# Autodesk Inventor assembly: Degrader_Assembly
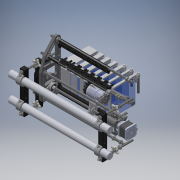
[picture p0: Inventor's stored thumbnail of the model, 180x180]
Saved by Autodesk Inventor 2019 (Build 230136000, 136)
## iProperties
Created: 2019-10-16
Part Number: Degrader_Assembly
Document SubType Name: Assembly
Designer: 19879326
Author: 19879326
## Documents named in this file (57)
- I:\Poster\CAD\CAD\Final\Degrader_Assembly.iam
- I:\Poster\CAD\CAD\Final\Mount\Mounting Rods.ipt
- I:\Poster\CAD\CAD\Final\Mount\Mount_Block.ipt
- I:\Poster\CAD\CAD\Final\Frame\Frame_Stepper_New.ipt
- I:\Poster\CAD\CAD\Final\Frame\Frame_Bearing_New.ipt
- I:\Poster\CAD\CAD\Final\Frame\Thread_Shaft_330mm.ipt
- I:\Poster\CAD\CAD\Final\Frame\300mm_Rod.ipt
- I:\Poster\CAD\CAD\Final\Mount\Mount_Thread.ipt
- I:\Poster\CAD\CAD\Final\Mount\M8_Nut.ipt
- I:\Poster\CAD\CAD\Final\Frame\Thread_Shaft_366mm.ipt
- I:\Poster\CAD\CAD\Final\Mount\Wing_Nut.ipt
- I:\Poster\CAD\CAD\Final\Mount\Frame_Mount.ipt
- I:\Poster\CAD\CAD\Final\Stepper Motor\Bearing.ipt
- I:\Poster\CAD\CAD\Final\Stepper Motor\Pillow_Stand.ipt
- I:\Poster\CAD\CAD\Final\Stepper Motor\Screw.ipt
- I:\Poster\CAD\CAD\Final\Stepper Motor\Stepper_Nema17.ipt
- I:\Poster\CAD\CAD\Final\Stepper Motor\Thread_Shaft.ipt
- I:\Poster\CAD\CAD\Final\Stepper Motor\Coupler.ipt
- I:\Poster\CAD\CAD\Final\DC motor\DC Gear.ipt
- I:\Poster\CAD\CAD\Final\DC motor\Frame_DC.ipt
- I:\Poster\CAD\CAD\Final\DC motor\Linear Bearing 8mm.ipt
- I:\Poster\CAD\CAD\Final\DC motor\DC_Motor.iam
- I:\Poster\CAD\CAD\Final\Sheet Holders\2mmFrame.ipt
- I:\Poster\CAD\CAD\Final\Sheet Holders\3mmFrame.ipt
- I:\Poster\CAD\CAD\Final\Sheet Holders\6mmFrame.ipt
- I:\Poster\CAD\CAD\Final\Sheet Holders\8mmFrame.ipt
- I:\Poster\CAD\CAD\Final\Sheet Holders\10mmFrame.ipt
- I:\Poster\CAD\CAD\Final\Sheet Holders\12mmFrame.ipt
- I:\Poster\CAD\CAD\Final\Sheet Holders\30mmFrame.ipt
- I:\Poster\CAD\CAD\Final\Sheet Holders\Spacer.ipt
- I:\Poster\CAD\CAD\Final\Switches\Roller_Switch._new.ipt
- I:\Poster\CAD\CAD\Final\Frame\M8_Nut.ipt
- I:\Poster\CAD\CAD\Final\Switches\30_Switch_Left.ipt
- I:\Poster\CAD\CAD\Final\Switches\30_Switch.ipt
- I:\Poster\CAD\CAD\Final\Switches\Switch holder_Right.ipt
- I:\Poster\CAD\CAD\Final\Switches\Switch holder_Left.ipt
- I:\Poster\CAD\CAD\Final\Switches\Roller_Spacer.ipt
- I:\Poster\CAD\CAD\Final\Switches\Roller_Spacer_P.ipt
- I:\Poster\CAD\CAD\Final\Switches\Roller_Switch _30_new.ipt
- I:\Poster\CAD\CAD\Final\Switches\Roller_Switch end.ipt
- I:\Poster\CAD\CAD\Final\Mount\Clamp_Mount.ipt
- I:\Poster\CAD\CAD\Final\Sheet Holders\Sheet_2mm.ipt
- I:\Poster\CAD\CAD\Final\Sheet Holders\Sheet_3mm.ipt
- I:\Poster\CAD\CAD\Final\Sheet Holders\Sheet_6mm.ipt
- I:\Poster\CAD\CAD\Final\Sheet Holders\Sheet_8mm.ipt
- I:\Poster\CAD\CAD\Final\Sheet Holders\Sheet_10mm.ipt
- I:\Poster\CAD\CAD\Final\Sheet Holders\Sheet_12mm.ipt
- I:\Poster\CAD\CAD\Final\Sheet Holders\Sheet_30mm.ipt
- I:\Poster\CAD\CAD\Final\Frame\Cap.ipt
- I:\Poster\CAD\CAD\Final\Sheet Holders\6mm Weight Clamp.ipt
- I:\Poster\CAD\CAD\Final\Sheet Holders\2mm_3mm Weight Clamp.ipt
- I:\Poster\CAD\CAD\Final\Sheet Holders\Weight_Thread_2mm.ipt
- I:\Poster\CAD\CAD\Final\Sheet Holders\Weight_Thread_3mm.ipt
- I:\Poster\CAD\CAD\Final\Sheet Holders\Weight_Thread_6mm.ipt
- I:\Poster\CAD\CAD\Final\Sheet Holders\frameClip.ipt
- I:\Poster\CAD\CAD\Final\DC motor\DC_Ring.ipt
- I:\Poster\CAD\CAD\Final\DC motor\Thread_Clip.ipt
## Components (143 placed, 55 different names)
1. Mounting Rods:1 — Mate:1, Mate:2, Mate:3, Flush:13, Mate:261, Mate:262, Mate:263, Mate:264
2. Mount_Block:1 — Mate:1, Flush:1, Mate:31, Mate:32, Mate:34, Mate:36, Mate:37, Mate:38, Mate:48, Mate:50, Flush:11, Flush:12, Flush:42, Flush:43, Mate:265
3. Mount_Block:2 — Mate:2, Mate:3, Flush:1, Mate:30, Mate:33, Mate:40, Mate:42, Mate:43, Mate:44, Mate:46, Mate:52, Flush:9, Flush:10, Flush:13, Flush:40, Flush:41
4. Frame_Bearing_New:1 — Mate:84, Mate:85, Mate:86, Mate:87, Mate:88, Flush:15, Flush:16, Flush:17, Flush:18, Flush:19, Mate:96, Mate:104, Mate:135, Mate:137, Mate:154, Mate:166, Mate:167, Mate:168, Mate:169, Mate:170, Mate:178, Mate:179, Mate:180, Mate:212, Mate:213, Mate:215, Mate:216, Mate:242, Angle:1, Mate:280, Mate:281, Mate:282, Mate:284, Mate:288
5. Frame_Stepper_New:1 — Mate:89, Mate:91, Mate:92, Mate:93, Mate:94, Mate:95, Mate:96, Mate:97, Mate:98, Mate:99, Mate:100, Mate:101, Mate:122, Mate:123, Mate:124, Mate:129, Mate:130, Mate:131, Mate:163, Mate:164, Mate:171, Mate:172, Mate:175, Mate:181, Mate:182, Mate:183, Mate:184, Mate:185, Mate:186, Mate:188, Mate:190, Mate:192, Mate:194, Flush:39, Mate:286, Mate:287, Mate:289, Mate:290, Mate:291
6. Mount_Thread:1 — Mate:30, Mate:41, Mate:53, Flush:9, Mate:79, Mate:114
7. Mount_Thread:2 — Mate:31, Mate:35, Mate:51, Flush:12, Mate:77, Mate:107, Mate:118
8. Mount_Thread:3 — Mate:32, Mate:39, Mate:49, Flush:11, Mate:81, Mate:120
9. Mount_Thread:4 — Mate:33, Mate:45, Mate:47, Flush:10, Mate:83, Mate:108, Mate:116
10. M8_Nut:1 — Mate:52, Mate:53
11. M8_Nut:2 — Mate:37, Mate:38, Mate:39
12. M8_Nut:3 — Mate:43, Mate:44, Mate:45
13. M8_Nut:4 — Mate:46, Mate:47
14. M8_Nut:5 — Mate:40, Mate:41, Mate:42
15. M8_Nut:6 — Mate:34, Mate:35, Mate:36
16. M8_Nut:7 — Mate:48, Mate:49
17. M8_Nut:8 — Mate:50, Mate:51
18. M8_Nut:9 — Mate:73, Mate:74, Mate:75, Mate:81
19. Wing_Nut:1 — Mate:73, Mate:74, Mate:75, Mate:110
20. M8_Nut:10 — Mate:70, Mate:71, Mate:72, Mate:79
21. Wing_Nut:2 — Mate:70, Mate:71, Mate:72, Mate:111
22. M8_Nut:11 — Mate:67, Mate:68, Mate:69, Mate:83
23. Wing_Nut:3 — Mate:67, Mate:68, Mate:69, Mate:112
24. M8_Nut:12 — Mate:64, Mate:65, Mate:66, Mate:77
25. Wing_Nut:4 — Mate:64, Mate:65, Mate:66, Mate:109
26. Thread_Shaft_330mm:1 — Mate:86, Flush:15, Mate:91, Mate:93, Mate:195, Mate:200, Mate:201, Mate:204, Mate:211, Mate:229, Mate:230, Mate:231, Mate:232, Mate:233, Mate:234
27. Thread_Shaft_366mm:1 — Mate:88, Flush:17, Mate:94, Mate:102, Mate:105, Mate:187, Mate:197, Mate:207, Mate:210
28. Thread_Shaft_330mm:2 — Mate:85, Flush:18, Mate:92, Mate:193, Mate:199, Mate:203, Mate:205, Mate:241, Mate:243, Mate:246, Mate:249, Mate:250, Mate:251, Mate:252, Mate:253, Mate:259, Mate:332
29. Thread_Shaft_366mm:2 — Mate:87, Flush:19, Mate:95, Mate:103, Mate:106, Mate:191, Mate:198, Mate:202, Mate:206
30. Thread_Shaft_330mm:3 — Mate:84, Flush:16, Mate:89, Mate:189, Mate:196, Mate:208, Mate:209, Mate:214, Mate:217, Mate:218, Mate:219, Mate:220, Mate:221, Mate:222
31. 300mm_Rod:1 — Mate:97, Mate:99, Mate:155, Mate:156, Mate:157, Mate:158, Mate:159, Mate:160, Mate:161, Mate:162, Mate:285
32. 300mm_Rod:2 — Mate:98, Mate:100, Mate:146, Mate:283
33. Frame_Mount:1 — Mate:101, Mate:102, Mate:103, Mate:108, Mate:111, Mate:112, Mate:113, Mate:115, Mate:173, Mate:174
34. Frame_Mount:2 — Mate:104, Mate:105, Mate:106, Mate:107, Mate:109, Mate:110, Mate:117, Mate:119, Mate:176, Mate:177, Mate:265
35. M8_Nut:13 — Mate:113, Mate:114
36. M8_Nut:14 — Mate:119, Mate:120
37. M8_Nut:15 — Mate:115, Mate:116
38. M8_Nut:16 — Mate:117, Mate:118
39. Bearing:1 — Mate:132, Mate:133, Mate:134
40. Pillow_Stand:1 — Mate:129, Mate:130, Mate:131, Mate:132, Mate:133
41. Screw:1 — Mate:142, Mate:143, Mate:144, Mate:147
42. Stepper_Nema17:1 — Mate:122, Mate:123, Mate:124, Mate:125, Mate:126
43. Thread_Shaft:1 — Mate:127, Mate:128, Mate:134, Mate:136, Mate:147
44. Bearing:2 — Mate:135, Mate:136, Mate:137
45. Coupler:1 — Mate:125, Mate:126, Mate:127, Mate:128
46. DC Gear:1 — Mate:145, Flush:21
47. Frame_DC:1 — Mate:138, Flush:20, Mate:139, Mate:140, Mate:142, Mate:143, Mate:144, Mate:292
48. Linear Bearing 8mm:1 — Mate:138, Flush:20, Mate:146
49. DC_Motor:1 [sub-assembly] — Mate:139, Mate:140, Mate:145, Flush:21, Mate:292, Mate:331
50. 2mmFrame:1 — Mate:148, Mate:161, Flush:39, Flush:49, Mate:266, Mate:267, Flush:51, Mate:293, Mate:294, Angle:2, Mate:295, Mate:296, Angle:3, Flush:66, Flush:75, Flush:77, Flush:78
51. 3mmFrame:1 — Mate:148, Mate:149, Mate:160, Flush:48, Flush:49, Mate:268, Mate:269, Flush:52, Mate:297, Mate:298, Mate:299, Mate:300, Angle:4, Angle:5, Flush:67, Flush:76, Flush:79, Flush:80
52. 6mmFrame:1 — Mate:149, Mate:150, Mate:159, Flush:47, Flush:48, Mate:270, Mate:271, Flush:53, Mate:301, Mate:302, Angle:6, Mate:303, Mate:304, Angle:7, Mate:330, Flush:81, Flush:82
53. 8mmFrame:1 — Mate:150, Mate:151, Mate:158, Flush:46, Flush:47, Mate:272, Mate:273, Flush:54, Mate:329, Flush:68, Flush:72, Flush:83, Flush:84
54. 10mmFrame:1 — Mate:151, Mate:152, Mate:157, Flush:45, Flush:46, Mate:274, Mate:275, Flush:55, Mate:328, Flush:69, Flush:71, Flush:85, Flush:86
55. 12mmFrame:1 — Mate:152, Mate:153, Mate:156, Flush:44, Flush:45, Mate:276, Mate:277, Flush:56, Mate:327, Flush:70, Flush:73, Flush:87, Flush:88
56. 30mmFrame:1 — Mate:153, Mate:154, Mate:155, Flush:44, Mate:278, Mate:279, Flush:57, Flush:64, Mate:312, Flush:65, Mate:326, Flush:74
57. Spacer:1 — Mate:162, Mate:163, Mate:164
58. M8_Nut:17 — Mate:178, Mate:199
59. M8_Nut:18 — Mate:175, Mate:208
60. M8_Nut:19 — Mate:174, Mate:207
61. M8_Nut:20 — Mate:172, Mate:205
62. M8_Nut:21 — Mate:173, Mate:206
63. M8_Nut:22 — Mate:181, Mate:194, Mate:195
64. M8_Nut:23 — Mate:179, Mate:200
65. M8_Nut:24 — Mate:185, Mate:186, Mate:187
66. M8_Nut:25 — Mate:180, Mate:196
67. M8_Nut:26 — Mate:170, Mate:210
68. M8_Nut:27 — Mate:177, Mate:198
69. M8_Nut:28 — Mate:169, Mate:209
70. M8_Nut:29 — Mate:168, Mate:203
71. M8_Nut:30 — Mate:167, Mate:202
72. M8_Nut:31 — Mate:166, Mate:201
73. M8_Nut:32 — Mate:184, Mate:188, Mate:189
74. M8_Nut:33 — Mate:183, Mate:190, Mate:191
75. M8_Nut:34 — Mate:182, Mate:192, Mate:193
76. M8_Nut:35 — Mate:176, Mate:197
77. M8_Nut:36 — Mate:171, Mate:204
78. 30_Switch_Left:1 — Mate:211, Mate:212, Mate:213, Mate:235, Flush:32
79. 30_Switch:1 — Mate:214, Mate:215, Mate:216, Mate:223, Flush:27
80. Switch holder_Right:1 — Mate:221, Mate:226, Mate:227, Flush:23, Flush:24
81. Switch holder_Right:2 — Mate:220, Mate:228, Flush:22
82. Switch holder_Right:3 — Mate:222, Mate:225, Mate:226, Flush:24, Flush:25
83. Switch holder_Right:4 — Mate:219, Mate:227, Mate:228, Flush:22, Flush:23
84. Switch holder_Right:5 — Mate:218, Mate:224, Mate:225, Flush:25, Flush:26
85. Switch holder_Right:6 — Mate:217, Mate:223, Mate:224, Flush:26, Flush:27
86. Switch holder_Left:1 — Mate:229, Mate:235, Mate:236, Flush:31, Flush:32
87. Switch holder_Left:2 — Mate:230, Mate:236, Mate:237, Flush:30, Flush:31
88. Switch holder_Left:3 — Mate:231, Mate:237, Mate:238, Flush:29, Flush:30
89. Switch holder_Left:4 — Mate:232, Mate:238, Mate:239, Flush:29, Flush:50
90. Switch holder_Left:5 — Mate:233, Mate:239, Mate:240, Flush:28, Flush:50
91. Switch holder_Left:6 — Mate:234, Mate:240, Flush:28
92. Roller_Spacer:1 — Mate:241, Mate:242, Angle:1, Mate:244, Mate:245
93. Roller_Spacer_P:1 — Mate:243, Mate:244, Mate:245, Mate:247, Mate:248
94. Roller_Switch._new:2 — Mate:252, Mate:256, Mate:257, Flush:35, Flush:36
95. Roller_Switch._new:3 — Mate:251, Mate:255, Mate:256, Flush:34, Flush:35
96. Roller_Switch._new:4 — Mate:250, Mate:254, Mate:255, Flush:33, Flush:34
97. Roller_Switch._new:5 — Mate:249, Mate:257, Mate:258, Flush:36, Flush:37
98. Roller_Switch._new:6 — Mate:253, Mate:258, Mate:260, Flush:37, Flush:38
99. Roller_Switch _30_new:1 — Mate:246, Mate:247, Mate:248, Mate:254, Flush:33
100. Roller_Switch end:1 — Mate:259, Mate:260, Flush:38, Angle:8
101. Clamp_Mount:1 — Mate:261, Flush:41
102. Clamp_Mount:2 — Mate:262, Flush:42
103. Clamp_Mount:3 — Mate:263, Flush:40
104. Clamp_Mount:4 — Mate:264, Flush:43
105. Sheet_2mm:1 — Mate:266, Mate:267, Flush:51, Mate:318, Mate:319
106. Sheet_3mm:1 — Mate:268, Mate:269, Flush:52, Mate:317, Mate:323
107. Sheet_6mm:1 — Mate:270, Mate:271, Flush:53, Mate:316, Mate:325
108. Sheet_8mm:1 — Mate:272, Mate:273, Flush:54, Mate:315, Mate:322
109. Sheet_10mm:1 — Mate:274, Mate:275, Flush:55, Mate:314, Mate:324
110. Sheet_12mm:1 — Mate:276, Mate:277, Flush:56, Mate:313, Mate:321
111. Sheet_30mm:1 — Mate:278, Mate:279, Flush:57, Mate:311, Mate:320
112. Cap:1 — Mate:285, Mate:286, Mate:287
113. Cap:2 — Mate:280, Mate:281, Mate:282
114. Cap:3 — Mate:283, Mate:284, Mate:288
115. Cap:4 — Mate:289, Mate:290, Mate:291
116. 6mm Weight Clamp:1 — Mate:303, Mate:304, Angle:7, Mate:306, Flush:63
117. 6mm Weight Clamp:2 — Mate:301, Mate:302, Angle:6, Mate:305, Flush:60
118. 2mm_3mm Weight Clamp:1 — Mate:293, Mate:294, Angle:2, Mate:310, Flush:58
119. 2mm_3mm Weight Clamp:2 — Mate:295, Mate:296, Angle:3, Mate:309, Flush:61
120. 2mm_3mm Weight Clamp:3 — Mate:299, Mate:300, Angle:4, Mate:307, Flush:62
121. 2mm_3mm Weight Clamp:4 — Mate:297, Mate:298, Angle:5, Mate:308, Flush:59
122. Weight_Thread_2mm:1 — Mate:310, Flush:58
123. Weight_Thread_3mm:1 — Mate:307, Flush:62
124. Weight_Thread_6mm:1 — Mate:306, Flush:63
125. Weight_Thread_2mm:2 — Mate:309, Flush:61
126. Weight_Thread_3mm:2 — Mate:308, Flush:59
127. Weight_Thread_6mm:2 — Mate:305, Flush:60
128. frameClip:1 — Mate:311, Flush:64, Mate:312
129. frameClip:2 — Mate:313, Flush:87, Flush:88
130. frameClip:3 — Mate:319, Flush:66, Flush:75
131. frameClip:4 — Mate:320, Flush:65, Mate:326, Flush:74
132. frameClip:5 — Mate:316, Flush:81, Flush:82
133. frameClip:6 — Mate:322, Mate:329, Flush:68, Flush:72
134. frameClip:7 — Mate:321, Mate:327, Flush:70, Flush:73
135. frameClip:8 — Mate:324, Mate:328, Flush:69, Flush:71
136. frameClip:9 — Mate:314, Flush:85, Flush:86
137. frameClip:10 — Mate:317, Flush:79, Flush:80
138. frameClip:11 — Mate:323, Flush:67, Flush:76
139. frameClip:12 — Mate:325, Mate:330
140. frameClip:13 — Mate:315, Flush:83, Flush:84
141. frameClip:14 — Mate:318, Flush:77, Flush:78
142. DC_Ring:1 — Mate:331, Angle:8
143. Thread_Clip:1 — Mate:332
## Relationships (376: Mate 288, Flush 80, Angle 8)
- Mate:1: Mounting Rods:1 ↔ Mount_Block:1
- Mate:2: Mounting Rods:1 ↔ Mount_Block:2
- Mate:3: Mounting Rods:1 ↔ Mount_Block:2
- Flush:1: Mount_Block:1 ↔ Mount_Block:2
- Mate:30: Mount_Block:2 ↔ Mount_Thread:1
- Mate:31: Mount_Block:1 ↔ Mount_Thread:2
- Mate:32: Mount_Block:1 ↔ Mount_Thread:3
- Mate:33: Mount_Block:2 ↔ Mount_Thread:4
- Mate:34: Mount_Block:1 ↔ M8_Nut:6
- Mate:35: Mount_Thread:2 ↔ M8_Nut:6
- Mate:36: Mount_Block:1 ↔ M8_Nut:6
- Mate:37: Mount_Block:1 ↔ M8_Nut:2
- Mate:38: Mount_Block:1 ↔ M8_Nut:2
- Mate:39: Mount_Thread:3 ↔ M8_Nut:2
- Mate:40: Mount_Block:2 ↔ M8_Nut:5
- Mate:41: Mount_Thread:1 ↔ M8_Nut:5
- Mate:42: Mount_Block:2 ↔ M8_Nut:5
- Mate:43: Mount_Block:2 ↔ M8_Nut:3
- Mate:44: Mount_Block:2 ↔ M8_Nut:3
- Mate:45: Mount_Thread:4 ↔ M8_Nut:3
- Mate:46: Mount_Block:2 ↔ M8_Nut:4
- Mate:47: Mount_Thread:4 ↔ M8_Nut:4
- Mate:48: Mount_Block:1 ↔ M8_Nut:7
- Mate:49: Mount_Thread:3 ↔ M8_Nut:7
- Mate:50: Mount_Block:1 ↔ M8_Nut:8
- Mate:51: Mount_Thread:2 ↔ M8_Nut:8
- Mate:52: Mount_Block:2 ↔ M8_Nut:1
- Mate:53: Mount_Thread:1 ↔ M8_Nut:1
- Flush:9 (-10 mm): Mount_Block:2 ↔ Mount_Thread:1
- Flush:10 (-10 mm): Mount_Block:2 ↔ Mount_Thread:4
- Flush:11 (-10 mm): Mount_Block:1 ↔ Mount_Thread:3
- Flush:12 (-10 mm): Mount_Block:1 ↔ Mount_Thread:2
- Flush:13 (30 mm): Mounting Rods:1 ↔ Mount_Block:2
- Mate:64: M8_Nut:12 ↔ Wing_Nut:4
- Mate:65: M8_Nut:12 ↔ Wing_Nut:4
- Mate:66: M8_Nut:12 ↔ Wing_Nut:4
- Mate:67: M8_Nut:11 ↔ Wing_Nut:3
- Mate:68: M8_Nut:11 ↔ Wing_Nut:3
- Mate:69: M8_Nut:11 ↔ Wing_Nut:3
- Mate:70: M8_Nut:10 ↔ Wing_Nut:2
- Mate:71: M8_Nut:10 ↔ Wing_Nut:2
- Mate:72: M8_Nut:10 ↔ Wing_Nut:2
- Mate:73: M8_Nut:9 ↔ Wing_Nut:1
- Mate:74: M8_Nut:9 ↔ Wing_Nut:1
- Mate:75: M8_Nut:9 ↔ Wing_Nut:1
- Mate:77: Mount_Thread:2 ↔ M8_Nut:12
- Mate:79: Mount_Thread:1 ↔ M8_Nut:10
- Mate:81: Mount_Thread:3 ↔ M8_Nut:9
- Mate:83: Mount_Thread:4 ↔ M8_Nut:11
- Mate:84: Frame_Bearing_New:1 ↔ Thread_Shaft_330mm:3
- Mate:85: Frame_Bearing_New:1 ↔ Thread_Shaft_330mm:2
- Mate:86: Frame_Bearing_New:1 ↔ Thread_Shaft_330mm:1
- Mate:87: Frame_Bearing_New:1 ↔ Thread_Shaft_366mm:2
- Mate:88: Frame_Bearing_New:1 ↔ Thread_Shaft_366mm:1
- Flush:15 (-15.5 mm): Frame_Bearing_New:1 ↔ Thread_Shaft_330mm:1
- Flush:16 (-15.5 mm): Frame_Bearing_New:1 ↔ Thread_Shaft_330mm:3
- Flush:17 (-33.5 mm): Frame_Bearing_New:1 ↔ Thread_Shaft_366mm:1
- Flush:18 (-15.5 mm): Frame_Bearing_New:1 ↔ Thread_Shaft_330mm:2
- Flush:19 (-33.5 mm): Frame_Bearing_New:1 ↔ Thread_Shaft_366mm:2
- Mate:89: Frame_Stepper_New:1 ↔ Thread_Shaft_330mm:3
- Mate:91: Frame_Stepper_New:1 ↔ Thread_Shaft_330mm:1
- Mate:92: Frame_Stepper_New:1 ↔ Thread_Shaft_330mm:2
- Mate:93: Frame_Stepper_New:1 ↔ Thread_Shaft_330mm:1
- Mate:94: Frame_Stepper_New:1 ↔ Thread_Shaft_366mm:1
- Mate:95: Frame_Stepper_New:1 ↔ Thread_Shaft_366mm:2
- Mate:96 (279 mm): Frame_Bearing_New:1 ↔ Frame_Stepper_New:1
- Mate:97: Frame_Stepper_New:1 ↔ 300mm_Rod:1
- Mate:98: Frame_Stepper_New:1 ↔ 300mm_Rod:2
- Mate:99 (5 mm): Frame_Stepper_New:1 ↔ 300mm_Rod:1
- Mate:100 (5 mm): Frame_Stepper_New:1 ↔ 300mm_Rod:2
- Mate:101: Frame_Stepper_New:1 ↔ Frame_Mount:1
- Mate:102: Thread_Shaft_366mm:1 ↔ Frame_Mount:1
- Mate:103: Thread_Shaft_366mm:2 ↔ Frame_Mount:1
- Mate:104: Frame_Bearing_New:1 ↔ Frame_Mount:2
- Mate:105: Thread_Shaft_366mm:1 ↔ Frame_Mount:2
- Mate:106: Thread_Shaft_366mm:2 ↔ Frame_Mount:2
- Mate:107: Mount_Thread:2 ↔ Frame_Mount:2
- Mate:108: Mount_Thread:4 ↔ Frame_Mount:1
- Mate:109: Wing_Nut:4 ↔ Frame_Mount:2
- Mate:110: Wing_Nut:1 ↔ Frame_Mount:2
- Mate:111: Wing_Nut:2 ↔ Frame_Mount:1
- Mate:112: Wing_Nut:3 ↔ Frame_Mount:1
- Mate:113: Frame_Mount:1 ↔ M8_Nut:13
- Mate:114: Mount_Thread:1 ↔ M8_Nut:13
- Mate:115: Frame_Mount:1 ↔ M8_Nut:15
- Mate:116: Mount_Thread:4 ↔ M8_Nut:15
- Mate:117: Frame_Mount:2 ↔ M8_Nut:16
- Mate:118: Mount_Thread:2 ↔ M8_Nut:16
- Mate:119: Frame_Mount:2 ↔ M8_Nut:14
- Mate:120: Mount_Thread:3 ↔ M8_Nut:14
- Mate:122: Frame_Stepper_New:1 ↔ Stepper_Nema17:1
- Mate:123: Frame_Stepper_New:1 ↔ Stepper_Nema17:1
- Mate:124: Frame_Stepper_New:1 ↔ Stepper_Nema17:1
- Mate:125: Stepper_Nema17:1 ↔ Coupler:1
- Mate:126 (-13 mm): Stepper_Nema17:1 ↔ Coupler:1
- Mate:127: Thread_Shaft:1 ↔ Coupler:1
- Mate:128 (-12 mm): Thread_Shaft:1 ↔ Coupler:1
- Mate:129: Frame_Stepper_New:1 ↔ Pillow_Stand:1
- Mate:130: Frame_Stepper_New:1 ↔ Pillow_Stand:1
- Mate:131: Frame_Stepper_New:1 ↔ Pillow_Stand:1
- Mate:132: Bearing:1 ↔ Pillow_Stand:1
- Mate:133: Bearing:1 ↔ Pillow_Stand:1
- Mate:134: Bearing:1 ↔ Thread_Shaft:1
- Mate:135: Frame_Bearing_New:1 ↔ Bearing:2
- Mate:136: Thread_Shaft:1 ↔ Bearing:2
- Mate:137: Frame_Bearing_New:1 ↔ Bearing:2
- Mate:138: Frame_DC:1 ↔ Linear Bearing 8mm:1
- Flush:20: Frame_DC:1 ↔ Linear Bearing 8mm:1
- Mate:139: Frame_DC:1 ↔ DC_Motor:1
- Mate:140: Frame_DC:1 ↔ DC_Motor:1
- Mate:142: Screw:1 ↔ Frame_DC:1
- Mate:143: Screw:1 ↔ Frame_DC:1
- Mate:144: Screw:1 ↔ Frame_DC:1
- Mate:145: DC Gear:1 ↔ DC_Motor:1
- Flush:21: DC Gear:1 ↔ DC_Motor:1
- Mate:146: 300mm_Rod:2 ↔ Linear Bearing 8mm:1
- Mate:147: Screw:1 ↔ Thread_Shaft:1
- Mate:148: 2mmFrame:1 ↔ 3mmFrame:1
- Mate:149: 3mmFrame:1 ↔ 6mmFrame:1
- Mate:150: 6mmFrame:1 ↔ 8mmFrame:1
- Mate:151: 8mmFrame:1 ↔ 10mmFrame:1
- Mate:152: 10mmFrame:1 ↔ 12mmFrame:1
- Mate:153: 12mmFrame:1 ↔ 30mmFrame:1
- Mate:154: Frame_Bearing_New:1 ↔ 30mmFrame:1
- Mate:155: 300mm_Rod:1 ↔ 30mmFrame:1
- Mate:156: 300mm_Rod:1 ↔ 12mmFrame:1
- Mate:157: 300mm_Rod:1 ↔ 10mmFrame:1
- Mate:158: 300mm_Rod:1 ↔ 8mmFrame:1
- Mate:159: 300mm_Rod:1 ↔ 6mmFrame:1
- Mate:160: 300mm_Rod:1 ↔ 3mmFrame:1
- Mate:161: 300mm_Rod:1 ↔ 2mmFrame:1
- Mate:162: 300mm_Rod:1 ↔ Spacer:1
- Mate:163: Frame_Stepper_New:1 ↔ Spacer:1
- Mate:164: Frame_Stepper_New:1 ↔ Spacer:1
- Mate:166: Frame_Bearing_New:1 ↔ M8_Nut:31
- Mate:167: Frame_Bearing_New:1 ↔ M8_Nut:30
- Mate:168: Frame_Bearing_New:1 ↔ M8_Nut:29
- Mate:169: Frame_Bearing_New:1 ↔ M8_Nut:28
- Mate:170: Frame_Bearing_New:1 ↔ M8_Nut:26
- Mate:171: Frame_Stepper_New:1 ↔ M8_Nut:36
- Mate:172: Frame_Stepper_New:1 ↔ M8_Nut:20
- Mate:173: Frame_Mount:1 ↔ M8_Nut:21
- Mate:174: Frame_Mount:1 ↔ M8_Nut:19
- Mate:175: Frame_Stepper_New:1 ↔ M8_Nut:18
- Mate:176: Frame_Mount:2 ↔ M8_Nut:35
- Mate:177: Frame_Mount:2 ↔ M8_Nut:27
- Mate:178: Frame_Bearing_New:1 ↔ M8_Nut:17
- Mate:179: Frame_Bearing_New:1 ↔ M8_Nut:23
- Mate:180: Frame_Bearing_New:1 ↔ M8_Nut:25
- Mate:181: Frame_Stepper_New:1 ↔ M8_Nut:22
- Mate:182: Frame_Stepper_New:1 ↔ M8_Nut:34
- Mate:183: Frame_Stepper_New:1 ↔ M8_Nut:33
- Mate:184: Frame_Stepper_New:1 ↔ M8_Nut:32
- Mate:185: Frame_Stepper_New:1 ↔ M8_Nut:24
- Mate:186: Frame_Stepper_New:1 ↔ M8_Nut:24
- Mate:187: Thread_Shaft_366mm:1 ↔ M8_Nut:24
- Mate:188: Frame_Stepper_New:1 ↔ M8_Nut:32
- Mate:189: Thread_Shaft_330mm:3 ↔ M8_Nut:32
- Mate:190: Frame_Stepper_New:1 ↔ M8_Nut:33
- Mate:191: Thread_Shaft_366mm:2 ↔ M8_Nut:33
- Mate:192: Frame_Stepper_New:1 ↔ M8_Nut:34
- Mate:193: Thread_Shaft_330mm:2 ↔ M8_Nut:34
- Mate:194: Frame_Stepper_New:1 ↔ M8_Nut:22
- Mate:195: Thread_Shaft_330mm:1 ↔ M8_Nut:22
- Mate:196: Thread_Shaft_330mm:3 ↔ M8_Nut:25
- Mate:197: Thread_Shaft_366mm:1 ↔ M8_Nut:35
- Mate:198: Thread_Shaft_366mm:2 ↔ M8_Nut:27
- Mate:199: Thread_Shaft_330mm:2 ↔ M8_Nut:17
- Mate:200: Thread_Shaft_330mm:1 ↔ M8_Nut:23
- Mate:201: Thread_Shaft_330mm:1 ↔ M8_Nut:31
- Mate:202: Thread_Shaft_366mm:2 ↔ M8_Nut:30
- Mate:203: Thread_Shaft_330mm:2 ↔ M8_Nut:29
- Mate:204: Thread_Shaft_330mm:1 ↔ M8_Nut:36
- Mate:205: Thread_Shaft_330mm:2 ↔ M8_Nut:20
- Mate:206: Thread_Shaft_366mm:2 ↔ M8_Nut:21
- Mate:207: Thread_Shaft_366mm:1 ↔ M8_Nut:19
- Mate:208: Thread_Shaft_330mm:3 ↔ M8_Nut:18
- Mate:209: Thread_Shaft_330mm:3 ↔ M8_Nut:28
- Mate:210: Thread_Shaft_366mm:1 ↔ M8_Nut:26
- Mate:211: Thread_Shaft_330mm:1 ↔ 30_Switch_Left:1
- Mate:212: Frame_Bearing_New:1 ↔ 30_Switch_Left:1
- Mate:213: Frame_Bearing_New:1 ↔ 30_Switch_Left:1
- Mate:214: Thread_Shaft_330mm:3 ↔ 30_Switch:1
- Mate:215: Frame_Bearing_New:1 ↔ 30_Switch:1
- Mate:216: Frame_Bearing_New:1 ↔ 30_Switch:1
- Mate:217: Thread_Shaft_330mm:3 ↔ Switch holder_Right:6
- Mate:218: Thread_Shaft_330mm:3 ↔ Switch holder_Right:5
- Mate:219: Thread_Shaft_330mm:3 ↔ Switch holder_Right:4
- Mate:220: Thread_Shaft_330mm:3 ↔ Switch holder_Right:2
- Mate:221: Thread_Shaft_330mm:3 ↔ Switch holder_Right:1
- Mate:222: Thread_Shaft_330mm:3 ↔ Switch holder_Right:3
- Mate:223: 30_Switch:1 ↔ Switch holder_Right:6
- Mate:224: Switch holder_Right:5 ↔ Switch holder_Right:6
- Mate:225: Switch holder_Right:3 ↔ Switch holder_Right:5
- Mate:226: Switch holder_Right:1 ↔ Switch holder_Right:3
- Mate:227: Switch holder_Right:1 ↔ Switch holder_Right:4
- Mate:228: Switch holder_Right:2 ↔ Switch holder_Right:4
- Flush:22: Switch holder_Right:2 ↔ Switch holder_Right:4
- Flush:23: Switch holder_Right:1 ↔ Switch holder_Right:4
- Flush:24: Switch holder_Right:1 ↔ Switch holder_Right:3
- Flush:25: Switch holder_Right:3 ↔ Switch holder_Right:5
- Flush:26: Switch holder_Right:5 ↔ Switch holder_Right:6
- Flush:27: 30_Switch:1 ↔ Switch holder_Right:6
- Mate:229: Thread_Shaft_330mm:1 ↔ Switch holder_Left:1
- Mate:230: Thread_Shaft_330mm:1 ↔ Switch holder_Left:2
- Mate:231: Thread_Shaft_330mm:1 ↔ Switch holder_Left:3
- Mate:232: Thread_Shaft_330mm:1 ↔ Switch holder_Left:4
- Mate:233: Thread_Shaft_330mm:1 ↔ Switch holder_Left:5
- Mate:234: Thread_Shaft_330mm:1 ↔ Switch holder_Left:6
- Mate:235: 30_Switch_Left:1 ↔ Switch holder_Left:1
- Mate:236: Switch holder_Left:1 ↔ Switch holder_Left:2
- Mate:237: Switch holder_Left:2 ↔ Switch holder_Left:3
- Mate:238: Switch holder_Left:3 ↔ Switch holder_Left:4
- Mate:239: Switch holder_Left:4 ↔ Switch holder_Left:5
- Mate:240: Switch holder_Left:5 ↔ Switch holder_Left:6
- Flush:28: Switch holder_Left:5 ↔ Switch holder_Left:6
- Flush:29: Switch holder_Left:3 ↔ Switch holder_Left:4
- Flush:30: Switch holder_Left:2 ↔ Switch holder_Left:3
- Flush:31: Switch holder_Left:1 ↔ Switch holder_Left:2
- Flush:32: 30_Switch_Left:1 ↔ Switch holder_Left:1
- Mate:241: Thread_Shaft_330mm:2 ↔ Roller_Spacer:1
- Mate:242: Frame_Bearing_New:1 ↔ Roller_Spacer:1
- Angle:1 (180 deg): Frame_Bearing_New:1 ↔ Roller_Spacer:1
- Mate:243: Thread_Shaft_330mm:2 ↔ Roller_Spacer_P:1
- Mate:244: Roller_Spacer:1 ↔ Roller_Spacer_P:1
- Mate:245: Roller_Spacer:1 ↔ Roller_Spacer_P:1
- Mate:246: Thread_Shaft_330mm:2 ↔ Roller_Switch _30_new:1
- Mate:247: Roller_Spacer_P:1 ↔ Roller_Switch _30_new:1
- Mate:248: Roller_Spacer_P:1 ↔ Roller_Switch _30_new:1
- Mate:249: Thread_Shaft_330mm:2 ↔ Roller_Switch._new:5
- Mate:250: Thread_Shaft_330mm:2 ↔ Roller_Switch._new:4
- Mate:251: Thread_Shaft_330mm:2 ↔ Roller_Switch._new:3
- Mate:252: Thread_Shaft_330mm:2 ↔ Roller_Switch._new:2
- Mate:253: Thread_Shaft_330mm:2 ↔ Roller_Switch._new:6
- Mate:254: Roller_Switch._new:4 ↔ Roller_Switch _30_new:1
- Mate:255: Roller_Switch._new:3 ↔ Roller_Switch._new:4
- Mate:256: Roller_Switch._new:2 ↔ Roller_Switch._new:3
- Mate:257: Roller_Switch._new:2 ↔ Roller_Switch._new:5
- Mate:258: Roller_Switch._new:5 ↔ Roller_Switch._new:6
- Mate:259: Thread_Shaft_330mm:2 ↔ Roller_Switch end:1
- Mate:260: Roller_Switch._new:6 ↔ Roller_Switch end:1
- Flush:33: Roller_Switch._new:4 ↔ Roller_Switch _30_new:1
- Flush:34: Roller_Switch._new:3 ↔ Roller_Switch._new:4
- Flush:35: Roller_Switch._new:2 ↔ Roller_Switch._new:3
- Flush:36: Roller_Switch._new:2 ↔ Roller_Switch._new:5
- Flush:37: Roller_Switch._new:5 ↔ Roller_Switch._new:6
- Flush:38: Roller_Switch._new:6 ↔ Roller_Switch end:1
- Flush:39: Frame_Stepper_New:1 ↔ 2mmFrame:1
- Mate:261: Mounting Rods:1 ↔ Clamp_Mount:1
- Mate:262: Mounting Rods:1 ↔ Clamp_Mount:2
- Mate:263: Mounting Rods:1 ↔ Clamp_Mount:3
- Mate:264: Mounting Rods:1 ↔ Clamp_Mount:4
- Flush:40: Mount_Block:2 ↔ Clamp_Mount:3
- Flush:41: Mount_Block:2 ↔ Clamp_Mount:1
- Flush:42: Mount_Block:1 ↔ Clamp_Mount:2
- Flush:43: Mount_Block:1 ↔ Clamp_Mount:4
- Mate:265 (40 mm): Mount_Block:1 ↔ Frame_Mount:2
- Flush:44: 12mmFrame:1 ↔ 30mmFrame:1
- Flush:45: 10mmFrame:1 ↔ 12mmFrame:1
- Flush:46: 8mmFrame:1 ↔ 10mmFrame:1
- Flush:47: 6mmFrame:1 ↔ 8mmFrame:1
- Flush:48: 3mmFrame:1 ↔ 6mmFrame:1
- Flush:49: 2mmFrame:1 ↔ 3mmFrame:1
- Flush:50: Switch holder_Left:4 ↔ Switch holder_Left:5
- Mate:266: 2mmFrame:1 ↔ Sheet_2mm:1
- Mate:267: 2mmFrame:1 ↔ Sheet_2mm:1
- Flush:51: 2mmFrame:1 ↔ Sheet_2mm:1
- Mate:268: 3mmFrame:1 ↔ Sheet_3mm:1
- Mate:269: 3mmFrame:1 ↔ Sheet_3mm:1
- Flush:52: 3mmFrame:1 ↔ Sheet_3mm:1
- Mate:270: 6mmFrame:1 ↔ Sheet_6mm:1
- Mate:271: 6mmFrame:1 ↔ Sheet_6mm:1
- Flush:53: 6mmFrame:1 ↔ Sheet_6mm:1
- Mate:272: 8mmFrame:1 ↔ Sheet_8mm:1
- Mate:273: 8mmFrame:1 ↔ Sheet_8mm:1
- Flush:54: 8mmFrame:1 ↔ Sheet_8mm:1
- Mate:274: 10mmFrame:1 ↔ Sheet_10mm:1
- Mate:275: 10mmFrame:1 ↔ Sheet_10mm:1
- Flush:55: 10mmFrame:1 ↔ Sheet_10mm:1
- Mate:276: 12mmFrame:1 ↔ Sheet_12mm:1
- Mate:277: 12mmFrame:1 ↔ Sheet_12mm:1
- Flush:56: 12mmFrame:1 ↔ Sheet_12mm:1
- Mate:278: 30mmFrame:1 ↔ Sheet_30mm:1
- Mate:279: 30mmFrame:1 ↔ Sheet_30mm:1
- Flush:57: 30mmFrame:1 ↔ Sheet_30mm:1
- Mate:280: Frame_Bearing_New:1 ↔ Cap:2
- Mate:281: Frame_Bearing_New:1 ↔ Cap:2
- Mate:282: Frame_Bearing_New:1 ↔ Cap:2
- Mate:283: 300mm_Rod:2 ↔ Cap:3
- Mate:284: Frame_Bearing_New:1 ↔ Cap:3
- Mate:285: 300mm_Rod:1 ↔ Cap:1
- Mate:286: Frame_Stepper_New:1 ↔ Cap:1
- Mate:287: Frame_Stepper_New:1 ↔ Cap:1
- Mate:288: Frame_Bearing_New:1 ↔ Cap:3
- Mate:289: Frame_Stepper_New:1 ↔ Cap:4
- Mate:290: Frame_Stepper_New:1 ↔ Cap:4
- Mate:291: Frame_Stepper_New:1 ↔ Cap:4
- Mate:292: Frame_DC:1 ↔ DC_Motor:1
- Mate:293: 2mmFrame:1 ↔ 2mm_3mm Weight Clamp:1
- Mate:294: 2mmFrame:1 ↔ 2mm_3mm Weight Clamp:1
- Angle:2 (180 deg): 2mmFrame:1 ↔ 2mm_3mm Weight Clamp:1
- Mate:295: 2mmFrame:1 ↔ 2mm_3mm Weight Clamp:2
- Mate:296: 2mmFrame:1 ↔ 2mm_3mm Weight Clamp:2
- Angle:3 (0 deg): 2mmFrame:1 ↔ 2mm_3mm Weight Clamp:2
- Mate:297: 3mmFrame:1 ↔ 2mm_3mm Weight Clamp:4
- Mate:298: 3mmFrame:1 ↔ 2mm_3mm Weight Clamp:4
- Mate:299: 3mmFrame:1 ↔ 2mm_3mm Weight Clamp:3
- Mate:300: 3mmFrame:1 ↔ 2mm_3mm Weight Clamp:3
- Angle:4 (180 deg): 3mmFrame:1 ↔ 2mm_3mm Weight Clamp:3
- Angle:5 (180 deg): 3mmFrame:1 ↔ 2mm_3mm Weight Clamp:4
- Mate:301: 6mmFrame:1 ↔ 6mm Weight Clamp:2
- Mate:302: 6mmFrame:1 ↔ 6mm Weight Clamp:2
- Angle:6 (180 deg): 6mmFrame:1 ↔ 6mm Weight Clamp:2
- Mate:303: 6mmFrame:1 ↔ 6mm Weight Clamp:1
- Mate:304: 6mmFrame:1 ↔ 6mm Weight Clamp:1
- Angle:7 (180 deg): 6mmFrame:1 ↔ 6mm Weight Clamp:1
- Mate:305: 6mm Weight Clamp:2 ↔ Weight_Thread_6mm:2
- Mate:306: 6mm Weight Clamp:1 ↔ Weight_Thread_6mm:1
- Mate:307: 2mm_3mm Weight Clamp:3 ↔ Weight_Thread_3mm:1
- Mate:308: 2mm_3mm Weight Clamp:4 ↔ Weight_Thread_3mm:2
- Mate:309: 2mm_3mm Weight Clamp:2 ↔ Weight_Thread_2mm:2
- Mate:310: 2mm_3mm Weight Clamp:1 ↔ Weight_Thread_2mm:1
- Flush:58 (-2 mm): 2mm_3mm Weight Clamp:1 ↔ Weight_Thread_2mm:1
- Flush:59 (-2 mm): 2mm_3mm Weight Clamp:4 ↔ Weight_Thread_3mm:2
- Flush:60 (2 mm): 6mm Weight Clamp:2 ↔ Weight_Thread_6mm:2
- Flush:61 (-2 mm): 2mm_3mm Weight Clamp:2 ↔ Weight_Thread_2mm:2
- Flush:62 (-2 mm): 2mm_3mm Weight Clamp:3 ↔ Weight_Thread_3mm:1
- Flush:63 (2 mm): 6mm Weight Clamp:1 ↔ Weight_Thread_6mm:1
- Mate:311: Sheet_30mm:1 ↔ frameClip:1
- Flush:64: 30mmFrame:1 ↔ frameClip:1
- Mate:312: 30mmFrame:1 ↔ frameClip:1
- Mate:313: Sheet_12mm:1 ↔ frameClip:2
- Mate:314: Sheet_10mm:1 ↔ frameClip:9
- Mate:315: Sheet_8mm:1 ↔ frameClip:13
- Mate:316: Sheet_6mm:1 ↔ frameClip:5
- Mate:317: Sheet_3mm:1 ↔ frameClip:10
- Mate:318: Sheet_2mm:1 ↔ frameClip:14
- Mate:319: Sheet_2mm:1 ↔ frameClip:3
- Mate:320: Sheet_30mm:1 ↔ frameClip:4
- Mate:321: Sheet_12mm:1 ↔ frameClip:7
- Mate:322: Sheet_8mm:1 ↔ frameClip:6
- Mate:323: Sheet_3mm:1 ↔ frameClip:11
- Mate:324: Sheet_10mm:1 ↔ frameClip:8
- Mate:325: Sheet_6mm:1 ↔ frameClip:12
- Flush:65: 30mmFrame:1 ↔ frameClip:4
- Mate:326: 30mmFrame:1 ↔ frameClip:4
- Mate:327: 12mmFrame:1 ↔ frameClip:7
- Mate:328: 10mmFrame:1 ↔ frameClip:8
- Mate:329: 8mmFrame:1 ↔ frameClip:6
- Mate:330: 6mmFrame:1 ↔ frameClip:12
- Flush:66: 2mmFrame:1 ↔ frameClip:3
- Flush:67: 3mmFrame:1 ↔ frameClip:11
- Flush:68: 8mmFrame:1 ↔ frameClip:6
- Flush:69: 10mmFrame:1 ↔ frameClip:8
- Flush:70: 12mmFrame:1 ↔ frameClip:7
- Flush:71: 10mmFrame:1 ↔ frameClip:8
- Flush:72: 8mmFrame:1 ↔ frameClip:6
- Flush:73: 12mmFrame:1 ↔ frameClip:7
- Flush:74: 30mmFrame:1 ↔ frameClip:4
- Flush:75: 2mmFrame:1 ↔ frameClip:3
- Flush:76: 3mmFrame:1 ↔ frameClip:11
- Flush:77: 2mmFrame:1 ↔ frameClip:14
- Flush:78: 2mmFrame:1 ↔ frameClip:14
- Flush:79: 3mmFrame:1 ↔ frameClip:10
- Flush:80: 3mmFrame:1 ↔ frameClip:10
- Flush:81: 6mmFrame:1 ↔ frameClip:5
- Flush:82: 6mmFrame:1 ↔ frameClip:5
- Flush:83: 8mmFrame:1 ↔ frameClip:13
- Flush:84: 8mmFrame:1 ↔ frameClip:13
- Flush:85: 10mmFrame:1 ↔ frameClip:9
- Flush:86: 10mmFrame:1 ↔ frameClip:9
- Flush:87: 12mmFrame:1 ↔ frameClip:2
- Flush:88: 12mmFrame:1 ↔ frameClip:2
- Mate:331: DC_Motor:1 ↔ DC_Ring:1
- Angle:8 (0 deg): Roller_Switch end:1 ↔ DC_Ring:1
- Mate:332: Thread_Shaft_330mm:2 ↔ Thread_Clip:1
